# Autodesk Inventor assembly: 4DoF Manipulator Type 2
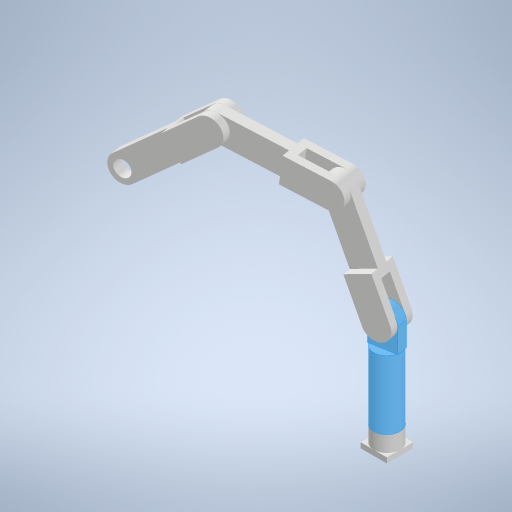
[picture p0: Inventor's stored thumbnail of the model, 512x512]
Saved by Autodesk Inventor 2023.2 (Build 272271030, 271C)
## iProperties
Created: 2023-06-26
Part Number: 4DoF Manipulator Type 2
Document SubType Name: Assembly
Designer: fist5
Author: fist5
## Documents named in this file (4)
- C:\Users\fist5\Desktop\4DoF Manipulator Type 2.iam
- C:\Users\fist5\Desktop\Manipulator Base Type2.ipt
- C:\Users\fist5\Desktop\Manipulator Link Type 2.ipt
- C:\Users\fist5\Desktop\Manipulator Link Type 1.ipt
## Components (5 placed, 3 different names)
1. Manipulator Base Type2:1 — Mate:1, Mate:2
2. Manipulator Link Type 2:1 — Mate:1, Mate:2, Mate:7, Mate:8
3. Manipulator Link Type 1:1 — Mate:3, Mate:6, Mate:7, Mate:8
4. Manipulator Link Type 1:2 — Mate:3, Mate:4, Mate:5, Mate:6
5. Manipulator Link Type 1:3 — Mate:4, Mate:5
## Relationships (8: Mate 8)
- Mate:1: Manipulator Base Type2:1 ↔ Manipulator Link Type 2:1
- Mate:2: Manipulator Base Type2:1 ↔ Manipulator Link Type 2:1
- Mate:3: Manipulator Link Type 1:1 ↔ Manipulator Link Type 1:2
- Mate:4: Manipulator Link Type 1:2 ↔ Manipulator Link Type 1:3
- Mate:5: Manipulator Link Type 1:2 ↔ Manipulator Link Type 1:3
- Mate:6: Manipulator Link Type 1:1 ↔ Manipulator Link Type 1:2
- Mate:7: Manipulator Link Type 2:1 ↔ Manipulator Link Type 1:1
- Mate:8: Manipulator Link Type 2:1 ↔ Manipulator Link Type 1:1
